# Autodesk Inventor assembly: Crossbrace
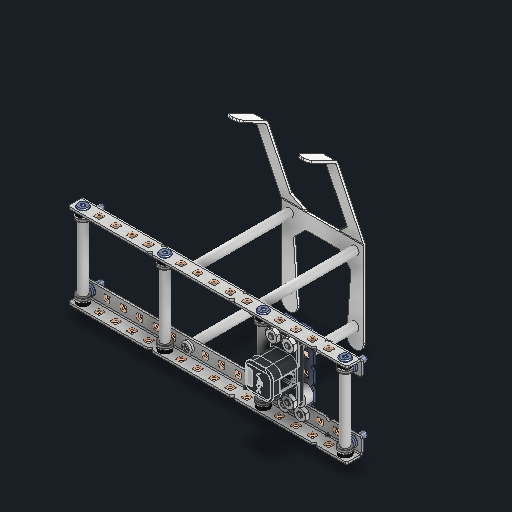
[picture p0: Inventor's stored thumbnail of the model, 512x512]
Saved by Autodesk Inventor 2025.1 (Build 291241000, 241)
## iProperties
Created: 2024-11-17
Part Number: Crossbrace
Document SubType Name: Assembly
Designer: avere
Author: avere
## Documents named in this file (23)
- C:\Users\avere\VEX\High Stakes\CAD\V3\Tower\Crossbrace.iam
- C:\Users\avere\VEX\High Stakes\CAD\ROBOPROS-CAD-Inventor\Structure\Angle\Aluminum 1x1\Alu Angle 1x1x17.ipt
- C:\Users\avere\VEX\High Stakes\CAD\ROBOPROS-CAD-Inventor\Structure\Nylon Standoff Rounded\Nylon Standoff 2.000.ipt
- C:\Users\avere\VEX\High Stakes\CAD\ROBOPROS-CAD-Inventor\Motion\Spacers\Spacer Nylon .375 OD\NSpacer .375 OD x .125.ipt
- C:\Users\avere\VEX\High Stakes\CAD\ROBOPROS-CAD-Inventor\Motion\Spacers\Spacer Nylon .375 OD.ipt
- C:\Users\avere\VEX\High Stakes\CAD\ROBOPROS-CAD-Inventor\Motion\Spacers\Washer Steel\SWasher .375 OD x .062500.ipt
- C:\Users\avere\VEX\High Stakes\CAD\ROBOPROS-CAD-Inventor\Motion\Spacers\Washer Steel.ipt
- C:\Users\avere\VEX\High Stakes\CAD\ROBOPROS-CAD-Inventor\Motion\Spacers\Washer Steel\SWasher .375 OD x .015625.ipt
- C:\Users\avere\VEX\High Stakes\CAD\ROBOPROS-CAD-Inventor\Motion\Spacers\Washer Steel\SWasher .375 OD x .031250.ipt
- C:\Users\avere\VEX\High Stakes\CAD\ROBOPROS-CAD-Inventor\Structure\Hardware\Screw Shoulder Robosource\SScrew Shoulder Smooth .500 x .04.ipt
- C:\Users\avere\VEX\High Stakes\CAD\ROBOPROS-CAD-Inventor\Structure\Hardware\Screw Shoulder Robosource.ipt
- C:\Users\avere\VEX\High Stakes\CAD\ROBOPROS-CAD-Inventor\Structure\Hardware\Screw Shoulder Robosource\SScrew Shoulder Smooth .375 x .12.ipt
- C:\Users\avere\VEX\High Stakes\CAD\ROBOPROS-CAD-Inventor\Motion\Spacers\Spacer Nylon .500 OD.ipt
- C:\Users\avere\VEX\High Stakes\CAD\V3\Tower\Color Sorter.iam
- C:\Users\avere\VEX\High Stakes\CAD\ROBOPROS-CAD-Inventor\Motion\Spacers\Spacer Nylon .500 OD\NSpacer White .500 OD x .125.ipt
- C:\Users\avere\VEX\High Stakes\CAD\ROBOPROS-CAD-Inventor\Motion\Spacers\Washer Steel\SWasher .500 OD x .062500\SWasher .500 OD x .062500.ipt
- C:\Users\avere\VEX\High Stakes\CAD\ROBOPROS-CAD-Inventor\Motion\Spacers\Washer Steel\SWasher .500 OD x .062500.ipt
- C:\Users\avere\VEX\High Stakes\CAD\ROBOPROS-CAD-Inventor\Structure\Hardware\Nut Nylon\Nut Nylon - White.ipt
- C:\Users\avere\VEX\High Stakes\CAD\ROBOPROS-CAD-Inventor\Structure\Hardware\Nut Nylon.ipt
- C:\Users\avere\VEX\High Stakes\CAD\ROBOPROS-CAD-Inventor\Structure\Hardware\Screw Nylon - Pan Head\NScrew Pan Head Threaded .625.ipt
- C:\Users\avere\VEX\High Stakes\CAD\V3\Tower\Custom Parts\Ring Guard.ipt
- C:\Users\avere\VEX\High Stakes\CAD\ROBOPROS-CAD-Inventor\Structure\Nylon Standoff Rounded\Nylon Standoff 3.000.ipt
- C:\Users\avere\VEX\High Stakes\CAD\ROBOPROS-CAD-Inventor\Structure\Hardware\Screw Nylon - Pan Head\NScrew Pan Head Threaded .250.ipt
## Components (76 placed, 16 different names)
1. Alu Angle 1x1x17:1 — Insert:37, Insert:46, Insert:47, Insert:52, Insert:57, Mate:3, Insert:61
2. Alu Angle 1x1x17:2 — Insert:35, Insert:36, Insert:48, Insert:50, Mate:2, Insert:58, Insert:64, Insert:65
3. Nylon Standoff 2.000:1
4. NSpacer .375 OD x .125:1
5. SWasher .375 OD x .062500:1
6. SWasher .375 OD x .015625:2
7. SWasher .375 OD x .031250:3
8. NSpacer .375 OD x .125:2
9. SWasher .375 OD x .062500:4
10. SWasher .375 OD x .015625:5
11. SWasher .375 OD x .031250:6
12. Nylon Standoff 2.000:2
13. NSpacer .375 OD x .125:3
14. SWasher .375 OD x .062500:7
15. SWasher .375 OD x .015625:8
16. SWasher .375 OD x .031250:9
17. NSpacer .375 OD x .125:4
18. SWasher .375 OD x .062500:10
19. SWasher .375 OD x .015625:11
20. SWasher .375 OD x .031250:12
21. SScrew Shoulder Smooth .500 x .04:1
22. SScrew Shoulder Smooth .500 x .04:2
23. SScrew Shoulder Smooth .500 x .04:3
24. SScrew Shoulder Smooth .500 x .04:4
25. SScrew Shoulder Smooth .375 x .12:5
26. SScrew Shoulder Smooth .375 x .12:6
27. SScrew Shoulder Smooth .375 x .12:7
28. SScrew Shoulder Smooth .375 x .12:8
29. Nylon Standoff 2.000:3
30. NSpacer .375 OD x .125:5
31. SWasher .375 OD x .062500:13
32. SWasher .375 OD x .015625:14
33. SWasher .375 OD x .031250:15
34. NSpacer .375 OD x .125:6 — Insert:35
35. SWasher .375 OD x .062500:16
36. SWasher .375 OD x .015625:17
37. SWasher .375 OD x .031250:18
38. SScrew Shoulder Smooth .500 x .04:9 — Insert:37
39. SScrew Shoulder Smooth .500 x .04:10 — Insert:36
40. Nylon Standoff 2.000:4
41. NSpacer .375 OD x .125:7 — Insert:46
42. SWasher .375 OD x .062500:19
43. SWasher .375 OD x .015625:20
44. SWasher .375 OD x .031250:21
45. NSpacer .375 OD x .125:8
46. SWasher .375 OD x .062500:22
47. SWasher .375 OD x .015625:23
48. SWasher .375 OD x .031250:24
49. SScrew Shoulder Smooth .500 x .04:11 — Insert:47
50. SScrew Shoulder Smooth .500 x .04:12 — Insert:48
51. Color Sorter:1 [sub-assembly] — Insert:50, Mate:2, Insert:53, Insert:54, Insert:62, Insert:63
52. Ring Guard:1 — Insert:55, Insert:56, Insert:59, Insert:60
53. Nylon Standoff 3.000:1 — Insert:55, Insert:57
54. Nylon Standoff 3.000:2 — Insert:56, Mate:3
55. Nylon Standoff 3.000:3 — Insert:58
56. Nylon Standoff 3.000:4 — Insert:59
57. NScrew Pan Head Threaded .250:9 — Insert:62
58. NScrew Pan Head Threaded .250:10 — Insert:63
59. Nut Nylon - White:3 — Insert:64
60. Nut Nylon - White:4 — Insert:65
61. Nut Nylon - White:1 — Insert:54
62. NScrew Pan Head Threaded .625:1 — Insert:53
63. SWasher .500 OD x .062500:1 — Insert:51
64. NSpacer White .500 OD x .125:1 — Insert:51, Insert:52
65. Nut Nylon - White:2
66. NScrew Pan Head Threaded .625:2
67. SWasher .500 OD x .062500:2
68. NSpacer White .500 OD x .125:2
69. NScrew Pan Head Threaded .250:1 — Insert:60
70. NScrew Pan Head Threaded .250:2
71. NScrew Pan Head Threaded .250:3
72. NScrew Pan Head Threaded .250:4
73. NScrew Pan Head Threaded .250:5 — Insert:61
74. NScrew Pan Head Threaded .250:6
75. NScrew Pan Head Threaded .250:7
76. NScrew Pan Head Threaded .250:8
## Component patterns: (2 elements, first: Nut Nylon - White:1 + NScrew Pan Head Threaded .625:1 + SWasher .500 OD x .062500:1 + NSpacer White .500 OD x .125:1), (4 elements, first: NScrew Pan Head Threaded .250:1), (4 elements, first: NScrew Pan Head Threaded .250:5)
## Relationships (66: Insert 64, Mate 2)
- [Insert]: NSpacer .375 OD x .125:1 ↔ SWasher .375 OD x .031250:3
- [Insert]: SWasher .375 OD x .062500:1 ↔ SWasher .375 OD x .031250:3
- [Insert]: SWasher .375 OD x .062500:1 ↔ SWasher .375 OD x .015625:2
- [Insert]: Nylon Standoff 2.000:1 ↔ SWasher .375 OD x .015625:2
- [Insert]: NSpacer .375 OD x .125:2 ↔ SWasher .375 OD x .031250:6
- [Insert]: SWasher .375 OD x .062500:4 ↔ SWasher .375 OD x .031250:6
- [Insert]: SWasher .375 OD x .062500:4 ↔ SWasher .375 OD x .015625:5
- [Insert]: Nylon Standoff 2.000:1 ↔ SWasher .375 OD x .015625:5
- [Insert]: NSpacer .375 OD x .125:3 ↔ SWasher .375 OD x .031250:9
- [Insert]: SWasher .375 OD x .062500:7 ↔ SWasher .375 OD x .031250:9
- [Insert]: SWasher .375 OD x .062500:7 ↔ SWasher .375 OD x .015625:8
- [Insert]: Nylon Standoff 2.000:2 ↔ SWasher .375 OD x .015625:8
- [Insert]: NSpacer .375 OD x .125:4 ↔ SWasher .375 OD x .031250:12
- [Insert]: SWasher .375 OD x .062500:10 ↔ SWasher .375 OD x .031250:12
- [Insert]: SWasher .375 OD x .062500:10 ↔ SWasher .375 OD x .015625:11
- [Insert]: Nylon Standoff 2.000:2 ↔ SWasher .375 OD x .015625:11
- [Insert]: Alu Angle 1x1x17:2 ↔ NSpacer .375 OD x .125:2
- [Insert]: Alu Angle 1x1x17:2 ↔ NSpacer .375 OD x .125:3
- [Insert]: Alu Angle 1x1x17:1 ↔ SScrew Shoulder Smooth .500 x .04:2
- [Insert]: Alu Angle 1x1x17:1 ↔ SScrew Shoulder Smooth .500 x .04:1
- [Insert]: Alu Angle 1x1x17:2 ↔ SScrew Shoulder Smooth .500 x .04:3
- [Insert]: Alu Angle 1x1x17:2 ↔ SScrew Shoulder Smooth .500 x .04:4
- [Insert]: Alu Angle 1x1x17:2 ↔ SScrew Shoulder Smooth .375 x .12:6
- [Insert]: Alu Angle 1x1x17:1 ↔ SScrew Shoulder Smooth .375 x .12:5
- [Insert]: Alu Angle 1x1x17:2 ↔ SScrew Shoulder Smooth .375 x .12:8
- [Insert]: Alu Angle 1x1x17:1 ↔ SScrew Shoulder Smooth .375 x .12:7
- [Insert]: NSpacer .375 OD x .125:5 ↔ SWasher .375 OD x .031250:15
- [Insert]: SWasher .375 OD x .062500:13 ↔ SWasher .375 OD x .031250:15
- [Insert]: SWasher .375 OD x .062500:13 ↔ SWasher .375 OD x .015625:14
- [Insert]: Nylon Standoff 2.000:3 ↔ SWasher .375 OD x .015625:14
- [Insert]: NSpacer .375 OD x .125:6 ↔ SWasher .375 OD x .031250:18
- [Insert]: SWasher .375 OD x .062500:16 ↔ SWasher .375 OD x .031250:18
- [Insert]: SWasher .375 OD x .062500:16 ↔ SWasher .375 OD x .015625:17
- [Insert]: Nylon Standoff 2.000:3 ↔ SWasher .375 OD x .015625:17
- Insert:35: Alu Angle 1x1x17:2 ↔ NSpacer .375 OD x .125:6
- Insert:36: Alu Angle 1x1x17:2 ↔ SScrew Shoulder Smooth .500 x .04:10
- Insert:37: Alu Angle 1x1x17:1 ↔ SScrew Shoulder Smooth .500 x .04:9
- [Insert]: NSpacer .375 OD x .125:7 ↔ SWasher .375 OD x .031250:21
- [Insert]: SWasher .375 OD x .062500:19 ↔ SWasher .375 OD x .031250:21
- [Insert]: SWasher .375 OD x .062500:19 ↔ SWasher .375 OD x .015625:20
- [Insert]: Nylon Standoff 2.000:4 ↔ SWasher .375 OD x .015625:20
- [Insert]: NSpacer .375 OD x .125:8 ↔ SWasher .375 OD x .031250:24
- [Insert]: SWasher .375 OD x .062500:22 ↔ SWasher .375 OD x .031250:24
- [Insert]: SWasher .375 OD x .062500:22 ↔ SWasher .375 OD x .015625:23
- [Insert]: Nylon Standoff 2.000:4 ↔ SWasher .375 OD x .015625:23
- Insert:46: Alu Angle 1x1x17:1 ↔ NSpacer .375 OD x .125:7
- Insert:47: Alu Angle 1x1x17:1 ↔ SScrew Shoulder Smooth .500 x .04:11
- Insert:48: Alu Angle 1x1x17:2 ↔ SScrew Shoulder Smooth .500 x .04:12
- Insert:50: Alu Angle 1x1x17:2 ↔ Color Sorter:1
- Mate:2: Alu Angle 1x1x17:2 ↔ Color Sorter:1
- Insert:51: SWasher .500 OD x .062500:1 ↔ NSpacer White .500 OD x .125:1
- Insert:52: Alu Angle 1x1x17:1 ↔ NSpacer White .500 OD x .125:1
- Insert:53: Color Sorter:1 ↔ NScrew Pan Head Threaded .625:1
- Insert:54: Color Sorter:1 ↔ Nut Nylon - White:1
- Insert:55: Ring Guard:1 ↔ Nylon Standoff 3.000:1
- Insert:56: Ring Guard:1 ↔ Nylon Standoff 3.000:2
- Insert:57: Alu Angle 1x1x17:1 ↔ Nylon Standoff 3.000:1
- Mate:3: Alu Angle 1x1x17:1 ↔ Nylon Standoff 3.000:2
- Insert:58: Alu Angle 1x1x17:2 ↔ Nylon Standoff 3.000:3
- Insert:59: Ring Guard:1 ↔ Nylon Standoff 3.000:4
- Insert:60: Ring Guard:1 ↔ NScrew Pan Head Threaded .250:1
- Insert:61: Alu Angle 1x1x17:1 ↔ NScrew Pan Head Threaded .250:5
- Insert:62: Color Sorter:1 ↔ NScrew Pan Head Threaded .250:9
- Insert:63: Color Sorter:1 ↔ NScrew Pan Head Threaded .250:10
- Insert:64: Alu Angle 1x1x17:2 ↔ Nut Nylon - White:3
- Insert:65: Alu Angle 1x1x17:2 ↔ Nut Nylon - White:4
## Named parameters: d6_d13 = 0 mm, d7_d14 = 0 mm, d15_d13 = 0 mm, d16_d11 = 0 mm, d17_d12 = 0 mm, d11_d18 = 0 mm, d19_d13 = 0 mm, d20_d14 = 0 mm, d21_d15_d13 = 0 mm, d22_d16_d11 = 0 mm, d23_d17_d12 = 0 mm, d24_d18 = 0 mm, d25_d11 = 0 mm, d26_d12 = 0 mm, d26_d19_d13 = 0 mm, d33_d20_d14 = 0 mm, d38_d21_d15_d13 = 0 mm, d39_d22_d16_d11 = 0 mm, d40_d23_d17_d12 = 0 mm, d41_d24_d18 = 0 mm, d42_d25_d11 = 0 mm, d43_d26_d12 = 0 mm, d47_d26_d19_d13 = 0 mm, d48_d33_d20_d14 = 0 mm, d49_d38_d21_d15_d13 = 0 mm, d50_d39_d22_d16_d11 = 0 mm, d51_d40_d23_d17_d12 = 0 mm, d52_d41_d24_d18 = 0 mm, d53_d42_d25_d11 = 0 mm, d54_d43_d26_d12 = 0 mm
